# Autodesk Inventor assembly: spacers
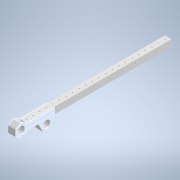
[picture p0: Inventor's stored thumbnail of the model, 180x180]
Saved by Autodesk Inventor 2020 (Build 240168000, 168)
## iProperties
Created: 2020-01-23
Part Number: spacers
Document SubType Name: Assembly
Designer: srini
Author: srini
## Documents named in this file (6)
- C:\Users\srini\Documents\FRC\2020\IntakeShooter\spacers.iam
- C:\Users\srini\Documents\FRC\2020\IntakeShooter\1x1x18.ipt
- C:\Users\srini\Documents\FRC\2020\IntakeShooter\VersaFrame_End_Bearing_Gusset_217-3554.ipt
- C:\Users\srini\Documents\FRC\2020\VersaFrame_Side_Bearing_Gusset_217-3553.ipt
- C:\Users\srini\Documents\FRC\2020\IntakeShooter\EndBearingMountSpacer.ipt
- C:\Users\srini\Documents\FRC\2020\IntakeShooter\SideSpacer.ipt
## Components (7 placed, 5 different names)
1. 1x1x18:1 — Insert:1, Insert:2, Insert:3, Insert:4, Insert:5, Insert:6, Insert:7, Insert:8
2. VersaFrame_End_Bearing_Gusset_217-3554:1 — Insert:1, Insert:2
3. VersaFrame_End_Bearing_Gusset_217-3554:2 — Insert:3, Insert:4, Flush:1
4. VersaFrame_Side_Bearing_Gusset_217-3553:1 — Insert:5, Insert:6
5. VersaFrame_Side_Bearing_Gusset_217-3553:2 — Insert:7, Insert:8, Flush:2
6. EndBearingMountSpacer:1 — Flush:1
7. SideSpacer:1 — Flush:2
## Relationships (10: Insert 8, Flush 2)
- Insert:1: 1x1x18:1 ↔ VersaFrame_End_Bearing_Gusset_217-3554:1
- Insert:2: 1x1x18:1 ↔ VersaFrame_End_Bearing_Gusset_217-3554:1
- Insert:3: 1x1x18:1 ↔ VersaFrame_End_Bearing_Gusset_217-3554:2
- Insert:4: 1x1x18:1 ↔ VersaFrame_End_Bearing_Gusset_217-3554:2
- Insert:5: 1x1x18:1 ↔ VersaFrame_Side_Bearing_Gusset_217-3553:1
- Insert:6: 1x1x18:1 ↔ VersaFrame_Side_Bearing_Gusset_217-3553:1
- Insert:7: 1x1x18:1 ↔ VersaFrame_Side_Bearing_Gusset_217-3553:2
- Insert:8: 1x1x18:1 ↔ VersaFrame_Side_Bearing_Gusset_217-3553:2
- Flush:1: VersaFrame_End_Bearing_Gusset_217-3554:2 ↔ EndBearingMountSpacer:1
- Flush:2: VersaFrame_Side_Bearing_Gusset_217-3553:2 ↔ SideSpacer:1
